# Autodesk Inventor assembly: ServoAndHorn
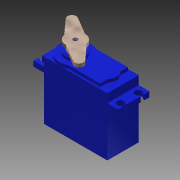
[picture p0: Inventor's stored thumbnail of the model, 180x180]
Saved by Autodesk Inventor 2014 SP1 (Build 180222100, 222)
## iProperties
Created: 2017-02-23
Part Number: ServoAndHorn
Document SubType Name: Assembly
Designer: danielsikar
Author: danielsikar
## Documents named in this file (3)
- C:\Users\danielsikar\Documents\Projects\iot-graffiti\cad\assemblies\ServoAndHorn.iam
- C:\Users\danielsikar\Documents\Arduino\IOT-Trike\Inventor\Parts\MG996RServo.ipt
- C:\Users\danielsikar\Documents\Arduino\IOT-Trike\Inventor\Parts\MG996RHorn.ipt
## Components (2 placed, 2 different names)
1. MG996RServo:1 — Flush:1, Flush:2, Flush:3, Mate:1, Mate:2
2. MG996RHorn:1 — Mate:1, Mate:2
## Relationships (5: Flush 3, Mate 2)
- Flush:1: MG996RServo:1
- Flush:2: MG996RServo:1
- Flush:3: MG996RServo:1
- Mate:1: MG996RServo:1 ↔ MG996RHorn:1
- Mate:2: MG996RServo:1 ↔ MG996RHorn:1
